# Autodesk Inventor assembly: Assembly of Conveyor Belt
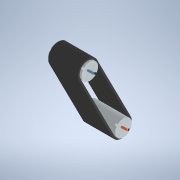
[picture p0: Inventor's stored thumbnail of the model, 180x180]
Saved by Autodesk Inventor 2022.2 (Build 262287000, 287)
## iProperties
Created: 2022-02-21
Part Number: Assembly of Conveyor Belt
Document SubType Name: Assembly
Designer: PRASHANTH
Author: PRASHANTH
## Documents named in this file (4)
- E:\BME\Autodesk Sample\Assembly of Conveyor Belt.iam
- E:\BME\Autodesk Sample\Conveyor Belt New.ipt
- E:\BME\Autodesk Sample\Conveyor Belt Shaft.ipt
- E:\BME\Autodesk Sample\Conveyor Shaft Pin.ipt
## Components (5 placed, 3 different names)
1. Conveyor Belt New:1 — Mate:1, Flush:1, Rotation/Translation:1, Mate:2, Flush:2
2. Conveyor Belt Shaft:1 — Mate:1, Flush:1, Rotation/Translation:1, Rotation:1, Mate:3, Flush:3
3. Conveyor Belt Shaft:2 — Rotation:1, Mate:2, Flush:2, Mate:4, Flush:4
4. Conveyor Shaft Pin:1 — Mate:3, Flush:3
5. Conveyor Shaft Pin:2 — Mate:4, Flush:4
## Relationships (10: Mate 4, Flush 4, RelateRotateTranslate 1, RelateRotation 1)
- Mate:1: Conveyor Belt New:1 ↔ Conveyor Belt Shaft:1
- Flush:1 (-5 mm): Conveyor Belt New:1 ↔ Conveyor Belt Shaft:1
- Rotation/Translation:1 [RelateRotateTranslate] (1 mm): Conveyor Belt New:1 ↔ Conveyor Belt Shaft:1
- Rotation:1 [RelateRotation] (1 ul): Conveyor Belt Shaft:1 ↔ Conveyor Belt Shaft:2
- Mate:2: Conveyor Belt New:1 ↔ Conveyor Belt Shaft:2
- Flush:2 (-5 mm): Conveyor Belt New:1 ↔ Conveyor Belt Shaft:2
- Mate:3: Conveyor Belt Shaft:1 ↔ Conveyor Shaft Pin:1
- Flush:3 (-10 mm): Conveyor Belt Shaft:1 ↔ Conveyor Shaft Pin:1
- Mate:4: Conveyor Belt Shaft:2 ↔ Conveyor Shaft Pin:2
- Flush:4 (-10 mm): Conveyor Belt Shaft:2 ↔ Conveyor Shaft Pin:2
